# Autodesk Inventor assembly: V-Wheel Kit
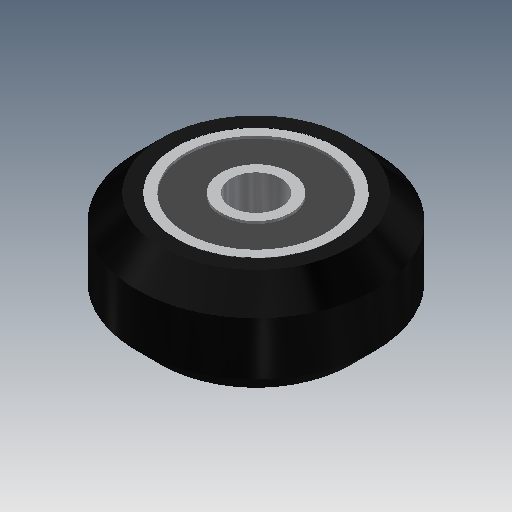
[picture p0: Inventor's stored thumbnail of the model, 512x512]
Saved by Autodesk Inventor 2020.3 (Build 243373000, 373)
## iProperties
Created: 2016-04-10
Part Number: V-Wheel Kit
Document SubType Name: Assembly
Designer: Ben
Author: Ben
## Documents named in this file (4)
- F:\UQ Engineering\2021 ~ 5th Year\Semester 2\METR4911-THESIS\FarmBot CAD\FarmBotV1\VSlotHardware\V-Wheel Kit.iam
- F:\UQ Engineering\2021 ~ 5th Year\Semester 2\METR4911-THESIS\FarmBot CAD\FarmBotV1\VSlotHardware\Solid V-Wheel.ipt
- F:\UQ Engineering\2021 ~ 5th Year\Semester 2\METR4911-THESIS\FarmBot CAD\FarmBotV1\VSlotHardware\Ball Bearing 625 2RS 5x16x5.ipt
- F:\UQ Engineering\2021 ~ 5th Year\Semester 2\METR4911-THESIS\FarmBot CAD\FarmBotV1\VSlotHardware\1mm 5mm shim.ipt
## Components (4 placed, 3 different names)
1. Solid V-Wheel:1 — Mate:1, Mate:2, Flush:1
2. Ball Bearing 625 2RS 5x16x5:1 — Mate:1, Mate:3, Mate:4, Mate:5
3. Ball Bearing 625 2RS 5x16x5:2 — Mate:2, Mate:3, Flush:1
4. 1mm 5mm shim:1 — Mate:4, Mate:5
## Relationships (6: Mate 5, Flush 1)
- Mate:1: Solid V-Wheel:1 ↔ Ball Bearing 625 2RS 5x16x5:1
- Mate:2: Solid V-Wheel:1 ↔ Ball Bearing 625 2RS 5x16x5:2
- Mate:3: Ball Bearing 625 2RS 5x16x5:1 ↔ Ball Bearing 625 2RS 5x16x5:2
- Flush:1: Solid V-Wheel:1 ↔ Ball Bearing 625 2RS 5x16x5:2
- Mate:4: Ball Bearing 625 2RS 5x16x5:1 ↔ 1mm 5mm shim:1
- Mate:5: Ball Bearing 625 2RS 5x16x5:1 ↔ 1mm 5mm shim:1
